# Autodesk Inventor assembly: assembly
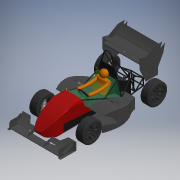
[picture p0: Inventor's stored thumbnail of the model, 180x180]
Saved by Autodesk Inventor 2018.2 (Build 222227000, 227)
## iProperties
Created: 2017-12-11
Part Number: assembly
Material: 一般
Document SubType Name: Assembly
Designer: kuwano
Author: kuwano
## Documents named in this file (8)
- Z:\各班フォルダ\2018\ボディ\カウル\AeroCAD2018\CAD\Inventor\製作用CAD\assembly.iam
- Z:\各班フォルダ\2018\ボディ\カウル\AeroCAD2018\CAD\Inventor\Assembly(KS-14.ver)\KS-14_SLow\KS-14_SLow_replace.iam
- Z:\各班フォルダ\2018\ボディ\カウル\AeroCAD2018\CAD\Inventor\製作用CAD\R-wing\R-wing.iam
- Z:\各班フォルダ\2018\ボディ\カウル\AeroCAD2018\CAD\Inventor\Aero Parts\F-wing\type7\F-wing.iam
- Z:\各班フォルダ\2018\ボディ\カウル\AeroCAD2018\CAD\Inventor\Aero Parts\Side Pontoon\type3(kuwano)\test.ipt
- Z:\各班フォルダ\2018\ボディ\カウル\AeroCAD2018\CAD\Inventor\Aero Parts\Side Pontoon\type3(kuwano)\defuser.ipt
- Z:\各班フォルダ\2018\ボディ\カウル\AeroCAD2018\CAD\Inventor\Aero Parts\Side Pontoon\type3(kuwano)\test_MIR.ipt
- Z:\各班フォルダ\2018\ボディ\カウル\AeroCAD2018\CAD\Inventor\Aero Parts\Side Pontoon\type3(kuwano)\defuser_MIR.ipt
## Components (7 placed, 7 different names)
1. KS-14_SLow_replace:1 [sub-assembly] — メイト:1, メイト:2, メイト:3
2. F-wing:1 [sub-assembly] — フラッシュ:2
3. R-wing:1 [sub-assembly] — フラッシュ:1, メイト:11
4. test:1 — メイト:4, メイト:5, メイト:6, フラッシュ:3, メイト:10
5. defuser:1 — メイト:4, メイト:5, メイト:6, フラッシュ:4
6. test_MIR:1 — メイト:7, メイト:8, メイト:9, フラッシュ:3, フラッシュ:5
7. defuser_MIR:1 — メイト:7, メイト:8, メイト:9, フラッシュ:4
## Relationships (16: Mate 11, Flush 5)
- メイト:1 [Mate]: KS-14_SLow_replace:1
- メイト:2 [Mate]: KS-14_SLow_replace:1
- メイト:3 [Mate]: KS-14_SLow_replace:1
- フラッシュ:1 [Flush]: R-wing:1
- フラッシュ:2 [Flush]: F-wing:1
- メイト:4 [Mate]: test:1 ↔ defuser:1
- メイト:5 [Mate]: test:1 ↔ defuser:1
- メイト:6 [Mate]: test:1 ↔ defuser:1
- メイト:7 [Mate]: test_MIR:1 ↔ defuser_MIR:1
- メイト:8 [Mate]: test_MIR:1 ↔ defuser_MIR:1
- メイト:9 [Mate]: test_MIR:1 ↔ defuser_MIR:1
- フラッシュ:3 [Flush]: test:1 ↔ test_MIR:1
- フラッシュ:4 [Flush]: defuser:1 ↔ defuser_MIR:1
- メイト:10 [Mate]: test:1
- フラッシュ:5 [Flush]: test_MIR:1
- メイト:11 [Mate] (500 mm): R-wing:1
